# Autodesk Inventor assembly: これで完成パネル型スカラアーム
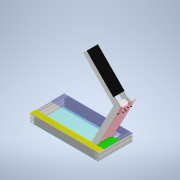
[picture p0: Inventor's stored thumbnail of the model, 180x180]
Saved by Autodesk Inventor 2022 (Build 260153000, 153)
## iProperties
Created: 2022-12-16
Part Number: これで完成パネル型スカラアーム
Document SubType Name: Assembly
Designer: tdn82
Author: tdn82
## Documents named in this file (28)
- C:\Users\tdn82\OneDrive\ドキュメント\Inventor\卒業研究パネル型スカラアーム\GrabCAD\panel-type-scalar-arm\パネル型スカラアーム\パネル型スカラアーム.iam
- C:\Users\tdn82\OneDrive\ドキュメント\Inventor\卒業研究パネル型スカラアーム\GrabCAD\panel-type-scalar-arm\パネル型スカラアーム\後ろカバー.ipt
- C:\Users\tdn82\OneDrive\ドキュメント\Inventor\卒業研究パネル型スカラアーム\GrabCAD\panel-type-scalar-arm\パネル型スカラアーム\HFS5-2040-180-Z5-YA10-YB99-YC170.ipt
- C:\Users\tdn82\OneDrive\ドキュメント\Inventor\卒業研究パネル型スカラアーム\GrabCAD\panel-type-scalar-arm\パネル型スカラアーム\HFS5-2040-320-TPW-Z5-YA42_5.ipt
- C:\Users\tdn82\OneDrive\ドキュメント\Inventor\卒業研究パネル型スカラアーム\GrabCAD\panel-type-scalar-arm\パネル型スカラアーム\HFS5-2040-320-TPW.ipt
- C:\Users\tdn82\OneDrive\ドキュメント\Inventor\卒業研究パネル型スカラアーム\GrabCAD\panel-type-scalar-arm\パネル型スカラアーム\HFS5-2040-180-Z5-YA10-YB170-Left.ipt
- C:\Users\tdn82\OneDrive\ドキュメント\Inventor\卒業研究パネル型スカラアーム\GrabCAD\panel-type-scalar-arm\パネル型スカラアーム\サーボ固定パーツ３Dプリンタ出力実験\サーボモータ固定用１軸目.ipt
- C:\Users\tdn82\OneDrive\ドキュメント\Inventor\卒業研究パネル型スカラアーム\GrabCAD\panel-type-scalar-arm\パネル型スカラアーム\サーボモータB3M1000_scale.ipt
- C:\Users\tdn82\OneDrive\ドキュメント\Inventor\卒業研究パネル型スカラアーム\GrabCAD\panel-type-scalar-arm\パネル型スカラアーム\サーボ固定パーツ３Dプリンタ出力実験\シャフト固定用.ipt
- C:\Users\tdn82\OneDrive\ドキュメント\Inventor\卒業研究パネル型スカラアーム\GrabCAD\panel-type-scalar-arm\パネル型スカラアーム\横長2ndフラットバー上 アルミフレーム用.ipt
- C:\Users\tdn82\OneDrive\ドキュメント\Inventor\卒業研究パネル型スカラアーム\GrabCAD\panel-type-scalar-arm\パネル型スカラアーム\横長2ndフラットバー下 アルミフレーム用.ipt
- C:\Users\tdn82\OneDrive\ドキュメント\Inventor\卒業研究パネル型スカラアーム\GrabCAD\panel-type-scalar-arm\パネル型スカラアーム\前カバー中盤左アーム固定.ipt
- C:\Users\tdn82\OneDrive\ドキュメント\Inventor\卒業研究パネル型スカラアーム\GrabCAD\panel-type-scalar-arm\パネル型スカラアーム\サーボ固定パーツ３Dプリンタ出力実験\サーボモータ固定用２軸目3mm改_new.ipt
- C:\Users\tdn82\OneDrive\ドキュメント\Inventor\卒業研究パネル型スカラアーム\GrabCAD\panel-type-scalar-arm\パネル型スカラアーム\アルミフリーホーン02137_AluminumFreeHornWithBearing_B3M_6000.ipt
- C:\Users\tdn82\OneDrive\ドキュメント\Inventor\卒業研究パネル型スカラアーム\GrabCAD\panel-type-scalar-arm\パネル型スカラアーム\シャフト.ipt
- C:\Users\tdn82\OneDrive\ドキュメント\Inventor\卒業研究パネル型スカラアーム\GrabCAD\panel-type-scalar-arm\パネル型スカラアーム\FL674ZZベアリング.ipt
- C:\Users\tdn82\OneDrive\ドキュメント\Inventor\卒業研究パネル型スカラアーム\GrabCAD\panel-type-scalar-arm\パネル型スカラアーム\シャフトカラー.ipt
- C:\Users\tdn82\OneDrive\ドキュメント\Inventor\卒業研究パネル型スカラアーム\GrabCAD\panel-type-scalar-arm\パネル型スカラアーム\横長3rdフラットバー下.ipt
- C:\Users\tdn82\OneDrive\ドキュメント\Inventor\卒業研究パネル型スカラアーム\GrabCAD\panel-type-scalar-arm\パネル型スカラアーム\CBE5-25.ipt
- C:\Users\tdn82\OneDrive\ドキュメント\Inventor\卒業研究パネル型スカラアーム\GrabCAD\panel-type-scalar-arm\パネル型スカラアーム\CBE5-20.ipt
- C:\Users\tdn82\OneDrive\ドキュメント\Inventor\卒業研究パネル型スカラアーム\GrabCAD\panel-type-scalar-arm\パネル型スカラアーム\CSPPN-ST-M2_6-18_203.ipt
- C:\Users\tdn82\OneDrive\ドキュメント\Inventor\卒業研究パネル型スカラアーム\GrabCAD\panel-type-scalar-arm\パネル型スカラアーム\CSPPN-STC-M3-6CSPPN-ST-M3-6_203.ipt
- C:\Users\tdn82\OneDrive\ドキュメント\Inventor\卒業研究パネル型スカラアーム\GrabCAD\panel-type-scalar-arm\パネル型スカラアーム\CSPPN-STC-M3-6CSPPN-ST-M3-10_203 - コピー.ipt
- C:\Users\tdn82\OneDrive\ドキュメント\Inventor\卒業研究パネル型スカラアーム\GrabCAD\panel-type-scalar-arm\パネル型スカラアーム\前下カバーサーボ隠し.ipt
- C:\Users\tdn82\OneDrive\ドキュメント\Inventor\卒業研究パネル型スカラアーム\GrabCAD\panel-type-scalar-arm\パネル型スカラアーム\前上カバーサーボ隠し.ipt
- C:\Users\tdn82\OneDrive\ドキュメント\Inventor\卒業研究パネル型スカラアーム\GrabCAD\panel-type-scalar-arm\パネル型スカラアーム\前カバー中段右.ipt
- C:\Users\tdn82\OneDrive\ドキュメント\Inventor\卒業研究パネル型スカラアーム\GrabCAD\panel-type-scalar-arm\パネル型スカラアーム\CSPPN-ST-M2_6-8_STEP_AP203AP214\CSPPN-ST-M2_6-8_203.ipt
- C:\Users\tdn82\OneDrive\ドキュメント\Inventor\卒業研究パネル型スカラアーム\GrabCAD\panel-type-scalar-arm\パネル型スカラアーム\三段目アクリル板.ipt
## Components (69 placed, 27 different names)
1. 後ろカバー:3 — メイト:1, メイト:2, フラッシュ:1, メイト:3, フラッシュ:2, フラッシュ:4, メイト:17, 挿入:66, 挿入:67, 挿入:68, 挿入:69
2. HFS5-2040-180-Z5-YA10-YB99-YC170:1 — メイト:3, フラッシュ:2, メイト:6, フラッシュ:4, メイト:9, フラッシュ:6, メイト:11, 挿入:26, 挿入:27, 挿入:28, 挿入:29, 挿入:30, 挿入:31, フラッシュ:9, メイト:18, フラッシュ:10, メイト:23, フラッシュ:11, メイト:25
3. HFS5-2040-320-TPW-Z5-YA42_5:1 — フラッシュ:9, メイト:18, フラッシュ:10, 挿入:32, 挿入:33, メイト:19, メイト:24, フラッシュ:14, メイト:27
4. HFS5-2040-320-TPW:1 — メイト:2, フラッシュ:1, メイト:6, メイト:16, フラッシュ:8
5. HFS5-2040-180-Z5-YA10-YB170-Left:1 — メイト:16, メイト:17, フラッシュ:8, 挿入:22, 挿入:23, 挿入:24, 挿入:25, フラッシュ:15
6. サーボモータ固定用１軸目:1 — メイト:9, フラッシュ:6, メイト:10, 挿入:1, 挿入:2, メイト:11, 挿入:34, 挿入:35, 挿入:36
7. サーボモータB3M1000_scale:1 — メイト:10, 挿入:1, 挿入:2, 挿入:12
8. サーボモータB3M1000_scale:2 — 挿入:18, 挿入:20, 挿入:37, 挿入:38, 挿入:72
9. シャフト固定用:1 — メイト:19, メイト:20, メイト:21, メイト:28
10. 横長2ndフラットバー上 アルミフレーム用:1 — 挿入:3, 挿入:4, 挿入:12
11. 横長2ndフラットバー下 アルミフレーム用:1 — 挿入:13, 挿入:14, 挿入:71
12. 前カバー中盤左アーム固定:1 — 挿入:3, 挿入:4, 挿入:7, 挿入:8, 挿入:13, 挿入:14, 挿入:42, 挿入:43, 挿入:44, 挿入:45, 挿入:46, 挿入:47, 挿入:48, 挿入:49, フラッシュ:12, メイト:26
13. サーボモータ固定用２軸目3mm改_new:1 — 挿入:7, 挿入:8, 挿入:37, 挿入:38, 挿入:39, 挿入:40, 挿入:41
14. アルミフリーホーン02137_AluminumFreeHornWithBearing_B3M_6000:1 — 挿入:18
15. シャフト:1 — メイト:27, メイト:28, メイト:30
16. FL674ZZベアリング:1 — 挿入:71, メイト:29
17. シャフトカラー:1 — メイト:29, メイト:30
18. 横長3rdフラットバー下:1 — 挿入:72, フラッシュ:16, 挿入:74
19. 横長3rdフラットバー下:2 — 挿入:20, フラッシュ:16, メイト:31, 挿入:73
20. CBE5-25:1 — 挿入:23
21. CBE5-25:2 — 挿入:22
22. CBE5-25:3 — 挿入:25
23. CBE5-25:4 — 挿入:24
24. CBE5-25:5 — 挿入:26
25. CBE5-25:6 — 挿入:27
26. CBE5-25:7 — 挿入:28
27. CBE5-25:8 — 挿入:29
28. CBE5-20:1 — 挿入:30
29. CBE5-20:2 — 挿入:31
30. CBE5-20:3 — 挿入:33, メイト:21
31. CBE5-20:4 — 挿入:32, メイト:20
32. CSPPN-ST-M2_6-18_203:1 — 挿入:34
33. CSPPN-ST-M2_6-18_203:2 — 挿入:35
34. CSPPN-ST-M2_6-18_203:3 — 挿入:36
35. CSPPN-ST-M2_6-18_203:4 — 挿入:39
36. CSPPN-ST-M2_6-18_203:5 — 挿入:41
37. CSPPN-ST-M2_6-18_203:6 — 挿入:40
38. CSPPN-STC-M3-6CSPPN-ST-M3-6_203:1 — 挿入:45
39. CSPPN-STC-M3-6CSPPN-ST-M3-6_203:2 — 挿入:42
40. CSPPN-STC-M3-6CSPPN-ST-M3-6_203:3 — 挿入:43
41. CSPPN-STC-M3-6CSPPN-ST-M3-6_203:4 — 挿入:44
42. CSPPN-STC-M3-6CSPPN-ST-M3-10_203 - コピー:1 — 挿入:76
43. CSPPN-STC-M3-6CSPPN-ST-M3-10_203 - コピー:2 — 挿入:75
44. CSPPN-STC-M3-6CSPPN-ST-M3-10_203 - コピー:3 — 挿入:78
45. CSPPN-STC-M3-6CSPPN-ST-M3-10_203 - コピー:4 — 挿入:77
46. CSPPN-STC-M3-6CSPPN-ST-M3-10_203 - コピー:5 — 挿入:49
47. CSPPN-STC-M3-6CSPPN-ST-M3-10_203 - コピー:6 — 挿入:48
48. CSPPN-STC-M3-6CSPPN-ST-M3-10_203 - コピー:7 — 挿入:47
49. CSPPN-STC-M3-6CSPPN-ST-M3-10_203 - コピー:8 — 挿入:46
50. CSPPN-ST-M2_6-8_203:1
51. CSPPN-ST-M2_6-8_203:2
52. CSPPN-ST-M2_6-8_203:3
53. CSPPN-ST-M2_6-8_203:4
54. CSPPN-ST-M2_6-8_203:5
55. CSPPN-ST-M2_6-8_203:6
56. CSPPN-ST-M2_6-8_203:7
57. CSPPN-ST-M2_6-8_203:8
58. CSPPN-ST-M2_6-8_203:9
59. CSPPN-ST-M2_6-8_203:10
60. CSPPN-ST-M2_6-8_203:11
61. CSPPN-ST-M2_6-8_203:12
62. CSPPN-STC-M3-6CSPPN-ST-M3-6_203:1 — 挿入:69
63. CSPPN-STC-M3-6CSPPN-ST-M3-6_203:2 — 挿入:68
64. CSPPN-STC-M3-6CSPPN-ST-M3-6_203:3 — 挿入:67
65. CSPPN-STC-M3-6CSPPN-ST-M3-6_203:4 — 挿入:66
66. 前下カバーサーボ隠し:1 — メイト:24, フラッシュ:13, フラッシュ:14
67. 前上カバーサーボ隠し:1 — メイト:25, メイト:26, フラッシュ:15
68. 前カバー中段右:1 — メイト:23, フラッシュ:11, フラッシュ:12, フラッシュ:13
69. 三段目アクリル板:1 — メイト:31, 挿入:73, 挿入:74, 挿入:75, 挿入:76, 挿入:77, 挿入:78
## Relationships (98: Insert 63, Mate 22, Flush 13)
- メイト:1 [Mate]: 後ろカバー:3
- メイト:2 [Mate]: 後ろカバー:3 ↔ HFS5-2040-320-TPW:1
- フラッシュ:1 [Flush]: 後ろカバー:3 ↔ HFS5-2040-320-TPW:1
- メイト:3 [Mate]: 後ろカバー:3 ↔ HFS5-2040-180-Z5-YA10-YB99-YC170:1
- フラッシュ:2 [Flush]: 後ろカバー:3 ↔ HFS5-2040-180-Z5-YA10-YB99-YC170:1
- メイト:6 [Mate]: HFS5-2040-180-Z5-YA10-YB99-YC170:1 ↔ HFS5-2040-320-TPW:1
- フラッシュ:4 [Flush]: 後ろカバー:3 ↔ HFS5-2040-180-Z5-YA10-YB99-YC170:1
- メイト:9 [Mate]: HFS5-2040-180-Z5-YA10-YB99-YC170:1 ↔ サーボモータ固定用１軸目:1
- フラッシュ:6 [Flush]: HFS5-2040-180-Z5-YA10-YB99-YC170:1 ↔ サーボモータ固定用１軸目:1
- メイト:10 [Mate]: サーボモータ固定用１軸目:1 ↔ サーボモータB3M1000_scale:1
- 挿入:1 [Insert]: サーボモータ固定用１軸目:1 ↔ サーボモータB3M1000_scale:1
- 挿入:2 [Insert]: サーボモータ固定用１軸目:1 ↔ サーボモータB3M1000_scale:1
- メイト:11 [Mate]: HFS5-2040-180-Z5-YA10-YB99-YC170:1 ↔ サーボモータ固定用１軸目:1
- 挿入:3 [Insert]: 横長2ndフラットバー上 アルミフレーム用:1 ↔ 前カバー中盤左アーム固定:1
- 挿入:4 [Insert]: 横長2ndフラットバー上 アルミフレーム用:1 ↔ 前カバー中盤左アーム固定:1
- 挿入:7 [Insert]: 前カバー中盤左アーム固定:1 ↔ サーボモータ固定用２軸目3mm改_new:1
- 挿入:8 [Insert]: 前カバー中盤左アーム固定:1 ↔ サーボモータ固定用２軸目3mm改_new:1
- 挿入:12 [Insert]: サーボモータB3M1000_scale:1 ↔ 横長2ndフラットバー上 アルミフレーム用:1
- 挿入:13 [Insert]: 横長2ndフラットバー下 アルミフレーム用:1 ↔ 前カバー中盤左アーム固定:1
- 挿入:14 [Insert]: 横長2ndフラットバー下 アルミフレーム用:1 ↔ 前カバー中盤左アーム固定:1
- 挿入:18 [Insert] (-1 mm): サーボモータB3M1000_scale:2 ↔ アルミフリーホーン02137_AluminumFreeHornWithBearing_B3M_6000:1
- 挿入:20 [Insert] (-1 mm): サーボモータB3M1000_scale:2 ↔ 横長3rdフラットバー下:2
- メイト:16 [Mate]: HFS5-2040-320-TPW:1 ↔ HFS5-2040-180-Z5-YA10-YB170-Left:1
- メイト:17 [Mate]: 後ろカバー:3 ↔ HFS5-2040-180-Z5-YA10-YB170-Left:1
- フラッシュ:8 [Flush]: HFS5-2040-320-TPW:1 ↔ HFS5-2040-180-Z5-YA10-YB170-Left:1
- 挿入:22 [Insert]: HFS5-2040-180-Z5-YA10-YB170-Left:1 ↔ CBE5-25:2
- 挿入:23 [Insert]: HFS5-2040-180-Z5-YA10-YB170-Left:1 ↔ CBE5-25:1
- 挿入:24 [Insert]: HFS5-2040-180-Z5-YA10-YB170-Left:1 ↔ CBE5-25:4
- 挿入:25 [Insert]: HFS5-2040-180-Z5-YA10-YB170-Left:1 ↔ CBE5-25:3
- 挿入:26 [Insert]: HFS5-2040-180-Z5-YA10-YB99-YC170:1 ↔ CBE5-25:5
- 挿入:27 [Insert]: HFS5-2040-180-Z5-YA10-YB99-YC170:1 ↔ CBE5-25:6
- 挿入:28 [Insert]: HFS5-2040-180-Z5-YA10-YB99-YC170:1 ↔ CBE5-25:7
- 挿入:29 [Insert]: HFS5-2040-180-Z5-YA10-YB99-YC170:1 ↔ CBE5-25:8
- 挿入:30 [Insert]: HFS5-2040-180-Z5-YA10-YB99-YC170:1 ↔ CBE5-20:1
- 挿入:31 [Insert]: HFS5-2040-180-Z5-YA10-YB99-YC170:1 ↔ CBE5-20:2
- フラッシュ:9 [Flush]: HFS5-2040-180-Z5-YA10-YB99-YC170:1 ↔ HFS5-2040-320-TPW-Z5-YA42_5:1
- メイト:18 [Mate]: HFS5-2040-180-Z5-YA10-YB99-YC170:1 ↔ HFS5-2040-320-TPW-Z5-YA42_5:1
- フラッシュ:10 [Flush]: HFS5-2040-180-Z5-YA10-YB99-YC170:1 ↔ HFS5-2040-320-TPW-Z5-YA42_5:1
- 挿入:32 [Insert]: HFS5-2040-320-TPW-Z5-YA42_5:1 ↔ CBE5-20:4
- 挿入:33 [Insert]: HFS5-2040-320-TPW-Z5-YA42_5:1 ↔ CBE5-20:3
- メイト:19 [Mate]: HFS5-2040-320-TPW-Z5-YA42_5:1 ↔ シャフト固定用:1
- メイト:20 [Mate]: シャフト固定用:1 ↔ CBE5-20:4
- メイト:21 [Mate]: シャフト固定用:1 ↔ CBE5-20:3
- 挿入:34 [Insert]: サーボモータ固定用１軸目:1 ↔ CSPPN-ST-M2_6-18_203:1
- 挿入:35 [Insert]: サーボモータ固定用１軸目:1 ↔ CSPPN-ST-M2_6-18_203:2
- 挿入:36 [Insert]: サーボモータ固定用１軸目:1 ↔ CSPPN-ST-M2_6-18_203:3
- 挿入:37 [Insert]: サーボモータB3M1000_scale:2 ↔ サーボモータ固定用２軸目3mm改_new:1
- 挿入:38 [Insert]: サーボモータB3M1000_scale:2 ↔ サーボモータ固定用２軸目3mm改_new:1
- 挿入:39 [Insert]: サーボモータ固定用２軸目3mm改_new:1 ↔ CSPPN-ST-M2_6-18_203:4
- 挿入:40 [Insert]: サーボモータ固定用２軸目3mm改_new:1 ↔ CSPPN-ST-M2_6-18_203:6
- 挿入:41 [Insert]: サーボモータ固定用２軸目3mm改_new:1 ↔ CSPPN-ST-M2_6-18_203:5
- 挿入:42 [Insert]: 前カバー中盤左アーム固定:1 ↔ CSPPN-STC-M3-6CSPPN-ST-M3-6_203:2
- 挿入:43 [Insert]: 前カバー中盤左アーム固定:1 ↔ CSPPN-STC-M3-6CSPPN-ST-M3-6_203:3
- 挿入:44 [Insert]: 前カバー中盤左アーム固定:1 ↔ CSPPN-STC-M3-6CSPPN-ST-M3-6_203:4
- 挿入:45 [Insert]: 前カバー中盤左アーム固定:1 ↔ CSPPN-STC-M3-6CSPPN-ST-M3-6_203:1
- 挿入:46 [Insert]: 前カバー中盤左アーム固定:1 ↔ CSPPN-STC-M3-6CSPPN-ST-M3-10_203 - コピー:8
- 挿入:47 [Insert]: 前カバー中盤左アーム固定:1 ↔ CSPPN-STC-M3-6CSPPN-ST-M3-10_203 - コピー:7
- 挿入:48 [Insert]: 前カバー中盤左アーム固定:1 ↔ CSPPN-STC-M3-6CSPPN-ST-M3-10_203 - コピー:6
- 挿入:49 [Insert]: 前カバー中盤左アーム固定:1 ↔ CSPPN-STC-M3-6CSPPN-ST-M3-10_203 - コピー:5
- [Insert]: 横長2ndフラットバー上 アルミフレーム用:1 ↔ CSPPN-ST-M2_6-8_203:1
- [Insert]: 横長2ndフラットバー上 アルミフレーム用:1 ↔ CSPPN-ST-M2_6-8_203:5
- [Insert]: 横長2ndフラットバー上 アルミフレーム用:1 ↔ CSPPN-ST-M2_6-8_203:6
- [Insert]: 横長2ndフラットバー上 アルミフレーム用:1 ↔ CSPPN-ST-M2_6-8_203:2
- [Insert]: 横長3rdフラットバー下:1 ↔ CSPPN-ST-M2_6-8_203:9
- [Insert]: 横長3rdフラットバー下:1 ↔ CSPPN-ST-M2_6-8_203:7
- [Insert]: 横長3rdフラットバー下:1 ↔ CSPPN-ST-M2_6-8_203:3
- [Insert]: 横長3rdフラットバー下:1 ↔ CSPPN-ST-M2_6-8_203:4
- [Insert]: 横長3rdフラットバー下:2 ↔ CSPPN-ST-M2_6-8_203:11
- [Insert]: 横長3rdフラットバー下:2 ↔ CSPPN-ST-M2_6-8_203:8
- [Insert]: 横長3rdフラットバー下:2 ↔ CSPPN-ST-M2_6-8_203:10
- [Insert]: 横長3rdフラットバー下:2 ↔ CSPPN-ST-M2_6-8_203:12
- 挿入:66 [Insert]: 後ろカバー:3 ↔ CSPPN-STC-M3-6CSPPN-ST-M3-6_203:4
- 挿入:67 [Insert]: 後ろカバー:3 ↔ CSPPN-STC-M3-6CSPPN-ST-M3-6_203:3
- 挿入:68 [Insert]: 後ろカバー:3 ↔ CSPPN-STC-M3-6CSPPN-ST-M3-6_203:2
- 挿入:69 [Insert]: 後ろカバー:3 ↔ CSPPN-STC-M3-6CSPPN-ST-M3-6_203:1
- メイト:23 [Mate]: HFS5-2040-180-Z5-YA10-YB99-YC170:1 ↔ 前カバー中段右:1
- フラッシュ:11 [Flush]: HFS5-2040-180-Z5-YA10-YB99-YC170:1 ↔ 前カバー中段右:1
- フラッシュ:12 [Flush]: 前カバー中盤左アーム固定:1 ↔ 前カバー中段右:1
- メイト:24 [Mate]: HFS5-2040-320-TPW-Z5-YA42_5:1 ↔ 前下カバーサーボ隠し:1
- フラッシュ:13 [Flush]: 前下カバーサーボ隠し:1 ↔ 前カバー中段右:1
- フラッシュ:14 [Flush]: HFS5-2040-320-TPW-Z5-YA42_5:1 ↔ 前下カバーサーボ隠し:1
- メイト:25 [Mate]: HFS5-2040-180-Z5-YA10-YB99-YC170:1 ↔ 前上カバーサーボ隠し:1
- メイト:26 [Mate]: 前カバー中盤左アーム固定:1 ↔ 前上カバーサーボ隠し:1
- フラッシュ:15 [Flush]: HFS5-2040-180-Z5-YA10-YB170-Left:1 ↔ 前上カバーサーボ隠し:1
- 挿入:71 [Insert]: 横長2ndフラットバー下 アルミフレーム用:1 ↔ FL674ZZベアリング:1
- メイト:27 [Mate]: HFS5-2040-320-TPW-Z5-YA42_5:1 ↔ シャフト:1
- メイト:28 [Mate]: シャフト固定用:1 ↔ シャフト:1
- メイト:29 [Mate]: FL674ZZベアリング:1 ↔ シャフトカラー:1
- メイト:30 [Mate]: シャフト:1 ↔ シャフトカラー:1
- 挿入:72 [Insert]: サーボモータB3M1000_scale:2 ↔ 横長3rdフラットバー下:1
- フラッシュ:16 [Flush]: 横長3rdフラットバー下:1 ↔ 横長3rdフラットバー下:2
- メイト:31 [Mate]: 横長3rdフラットバー下:2 ↔ 三段目アクリル板:1
- 挿入:73 [Insert]: 横長3rdフラットバー下:2 ↔ 三段目アクリル板:1
- 挿入:74 [Insert]: 横長3rdフラットバー下:1 ↔ 三段目アクリル板:1
- 挿入:75 [Insert]: CSPPN-STC-M3-6CSPPN-ST-M3-10_203 - コピー:2 ↔ 三段目アクリル板:1
- 挿入:76 [Insert]: CSPPN-STC-M3-6CSPPN-ST-M3-10_203 - コピー:1 ↔ 三段目アクリル板:1
- 挿入:77 [Insert]: CSPPN-STC-M3-6CSPPN-ST-M3-10_203 - コピー:4 ↔ 三段目アクリル板:1
- 挿入:78 [Insert]: CSPPN-STC-M3-6CSPPN-ST-M3-10_203 - コピー:3 ↔ 三段目アクリル板:1
